# Autodesk Inventor assembly: Full_Assembly
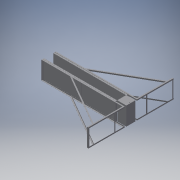
[picture p0: Inventor's stored thumbnail of the model, 180x180]
Saved by Autodesk Inventor 2017 (Build 210142000, 142)
## iProperties
Created: 2018-10-22
Part Number: Full_Assembly
Document SubType Name: Assembly
Designer: mcgratta
Author: mcgratta
## Documents named in this file (12)
- C:\Users\mcgratta\Documents\FDS_Validation_Test_Reports\FM_Parallel_Panels\Full_Assembly.iam
- C:\Users\mcgratta\Documents\FDS_Validation_Test_Reports\FM_Parallel_Panels\Angle_4-ft.ipt
- C:\Users\mcgratta\Documents\FDS_Validation_Test_Reports\FM_Parallel_Panels\Angle_9-ft.ipt
- C:\Users\mcgratta\Documents\FDS_Validation_Test_Reports\FM_Parallel_Panels\Right_Brace.ipt
- C:\Users\mcgratta\Documents\FDS_Validation_Test_Reports\FM_Parallel_Panels\Left_Brace.ipt
- C:\Users\mcgratta\Documents\FDS_Validation_Test_Reports\FM_Parallel_Panels\Angle_2-ft.ipt
- C:\Users\mcgratta\Documents\FDS_Validation_Test_Reports\FM_Parallel_Panels\Bar_2-ft.ipt
- C:\Users\mcgratta\Documents\FDS_Validation_Test_Reports\FM_Parallel_Panels\Right_Assembly.iam
- C:\Users\mcgratta\Documents\FDS_Validation_Test_Reports\FM_Parallel_Panels\Plywood.ipt
- C:\Users\mcgratta\Documents\FDS_Validation_Test_Reports\FM_Parallel_Panels\Marinite.ipt
- C:\Users\mcgratta\Documents\FDS_Validation_Test_Reports\FM_Parallel_Panels\Sample.ipt
- C:\Users\mcgratta\Documents\FDS_Validation_Test_Reports\FM_Parallel_Panels\Burner.ipt
## Components (19 placed, 11 different names)
1. Angle_4-ft:1 — Flush:1, Flush:2, Mate:1, Mate:4, Flush:5, Mate:8, Mate:9, Mate:11, Flush:6, Flush:8, Flush:9
2. Angle_4-ft:2 — Flush:1, Flush:2, Mate:1, Mate:3, Mate:7, Mate:12, Mate:17, Mate:18, Mate:19, Flush:25
3. Angle_9-ft:1 — Flush:3, Flush:4, Mate:2, Mate:3, Mate:5, Mate:6, Mate:15, Mate:16, Mate:20, Mate:22, Mate:27, Flush:16
4. Angle_9-ft:2 — Flush:3, Flush:4, Mate:2, Mate:4, Flush:5, Mate:10, Mate:13, Flush:7, Mate:14, Mate:21, Mate:24
5. Right_Brace:1 — Mate:5, Mate:6, Mate:7
6. Left_Brace:1 — Mate:8, Mate:9, Mate:10
7. Angle_2-ft:1 — Mate:11, Flush:6, Mate:12
8. Angle_2-ft:2 — Mate:13, Flush:7, Mate:14, Mate:23, Mate:24, Flush:12
9. Bar_2-ft:1 — Mate:21, Mate:22, Mate:23
10. Bar_2-ft:2 — Mate:17, Mate:18, Mate:20
11. Bar_2-ft:3 — Mate:15, Mate:16, Mate:19
12. Right_Assembly:1 [sub-assembly] — Flush:8, Flush:9, Flush:10, Mate:25, Flush:11, Flush:15, Flush:26, Mate:32
13. Plywood:1 — Flush:10, Mate:25, Flush:11, Flush:15, Mate:26, Mate:28, Flush:17, Flush:18
14. Plywood:2 — Flush:12, Mate:26, Mate:27, Flush:16, Flush:19, Mate:29, Flush:20
15. Marinite:1 — Flush:19, Mate:29, Flush:20, Mate:30, Flush:21, Flush:22
16. Marinite:2 — Mate:28, Flush:17, Flush:18, Flush:23, Flush:24, Mate:31
17. Sample:1 — Mate:30, Flush:21, Flush:22
18. Sample:2 — Flush:23, Flush:24, Mate:31
19. Burner:1 — Flush:25, Flush:26, Mate:32
## Relationships (56: Mate 32, Flush 24)
- Flush:1: Angle_4-ft:1 ↔ Angle_4-ft:2
- Flush:2: Angle_4-ft:1 ↔ Angle_4-ft:2
- Mate:1 (603.25 mm): Angle_4-ft:1 ↔ Angle_4-ft:2
- Flush:3: Angle_9-ft:1 ↔ Angle_9-ft:2
- Flush:4: Angle_9-ft:1 ↔ Angle_9-ft:2
- Mate:2 (596.9 mm): Angle_9-ft:1 ↔ Angle_9-ft:2
- Mate:3: Angle_4-ft:2 ↔ Angle_9-ft:1
- Mate:4: Angle_4-ft:1 ↔ Angle_9-ft:2
- Flush:5: Angle_4-ft:1 ↔ Angle_9-ft:2
- Mate:5: Angle_9-ft:1 ↔ Right_Brace:1
- Mate:6: Angle_9-ft:1 ↔ Right_Brace:1
- Mate:7: Angle_4-ft:2 ↔ Right_Brace:1
- Mate:8 (3.175 mm): Angle_4-ft:1 ↔ Left_Brace:1
- Mate:9: Angle_4-ft:1 ↔ Left_Brace:1
- Mate:10: Angle_9-ft:2 ↔ Left_Brace:1
- Mate:11: Angle_4-ft:1 ↔ Angle_2-ft:1
- Flush:6: Angle_4-ft:1 ↔ Angle_2-ft:1
- Mate:12: Angle_4-ft:2 ↔ Angle_2-ft:1
- Mate:13: Angle_9-ft:2 ↔ Angle_2-ft:2
- Flush:7: Angle_9-ft:2 ↔ Angle_2-ft:2
- Mate:14: Angle_9-ft:2 ↔ Angle_2-ft:2
- Mate:15: Angle_9-ft:1 ↔ Bar_2-ft:3
- Mate:16: Angle_9-ft:1 ↔ Bar_2-ft:3
- Mate:17: Angle_4-ft:2 ↔ Bar_2-ft:2
- Mate:18: Angle_4-ft:2 ↔ Bar_2-ft:2
- Mate:19 (304.8 mm): Angle_4-ft:2 ↔ Bar_2-ft:3
- Mate:20 (304.8 mm): Angle_9-ft:1 ↔ Bar_2-ft:2
- Mate:21: Angle_9-ft:2 ↔ Bar_2-ft:1
- Mate:22: Angle_9-ft:1 ↔ Bar_2-ft:1
- Mate:23 (1219.2 mm): Angle_2-ft:2 ↔ Bar_2-ft:1
- Mate:24: Angle_9-ft:2 ↔ Angle_2-ft:2
- Flush:8: Angle_4-ft:1 ↔ Right_Assembly:1
- Flush:9: Angle_4-ft:1 ↔ Right_Assembly:1
- Flush:10: Right_Assembly:1 ↔ Plywood:1
- Mate:25: Right_Assembly:1 ↔ Plywood:1
- Flush:11 (-12.7 mm): Right_Assembly:1 ↔ Plywood:1
- Flush:12: Angle_2-ft:2 ↔ Plywood:2
- Flush:15: Right_Assembly:1 ↔ Plywood:1
- Mate:26 (381 mm): Plywood:1 ↔ Plywood:2
- Mate:27: Angle_9-ft:1 ↔ Plywood:2
- Flush:16: Angle_9-ft:1 ↔ Plywood:2
- Mate:28: Plywood:1 ↔ Marinite:2
- Flush:17: Plywood:1 ↔ Marinite:2
- Flush:18: Plywood:1 ↔ Marinite:2
- Flush:19: Plywood:2 ↔ Marinite:1
- Mate:29: Plywood:2 ↔ Marinite:1
- Flush:20: Plywood:2 ↔ Marinite:1
- Mate:30: Marinite:1 ↔ Sample:1
- Flush:21: Marinite:1 ↔ Sample:1
- Flush:22: Marinite:1 ↔ Sample:1
- Flush:23: Marinite:2 ↔ Sample:2
- Flush:24: Marinite:2 ↔ Sample:2
- Mate:31: Marinite:2 ↔ Sample:2
- Flush:25: Angle_4-ft:2 ↔ Burner:1
- Flush:26: Right_Assembly:1 ↔ Burner:1
- Mate:32 (50.8 mm): Right_Assembly:1 ↔ Burner:1
